# Autodesk Inventor assembly: Montagem do revórví
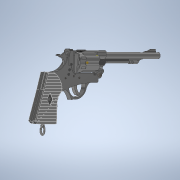
[picture p0: Inventor's stored thumbnail of the model, 180x180]
Saved by Autodesk Inventor 2021 (Build 250183000, 183)
## iProperties
Created: 2020-11-21
Part Number: Montagem do revórví
Document SubType Name: Assembly
Designer: Bruno
Author: Bruno
## Documents named in this file (20)
- C:\Users\Bruno\Documents\Quadirmestre Suplementar\Projeto Assistido por Computador\Novas peças revólver\Montagem do revórví.iam
- C:\Users\Bruno\Documents\Quadirmestre Suplementar\Projeto Assistido por Computador\Novas peças revólver\Part19.ipt
- C:\Users\Bruno\Documents\Quadirmestre Suplementar\Projeto Assistido por Computador\Novas peças revólver\Part22_1.ipt
- C:\Users\Bruno\Documents\Quadirmestre Suplementar\Projeto Assistido por Computador\Novas peças revólver\Part22_2.ipt
- C:\Users\Bruno\Documents\Quadirmestre Suplementar\Projeto Assistido por Computador\Novas peças revólver\Part35.ipt
- C:\Users\Bruno\Documents\Quadirmestre Suplementar\Projeto Assistido por Computador\Novas peças revólver\Montagem peças superiores.iam
- C:\Users\Bruno\Documents\Quadirmestre Suplementar\Projeto Assistido por Computador\Novas peças revólver\Montagem peças 11 a 14.iam
- C:\Users\Bruno\Documents\Quadirmestre Suplementar\Projeto Assistido por Computador\Novas peças revólver\Part6.ipt
- C:\Users\Bruno\Documents\Quadirmestre Suplementar\Projeto Assistido por Computador\Novas peças revólver\Montagem peças internas.iam
- C:\Users\Bruno\Documents\Quadirmestre Suplementar\Projeto Assistido por Computador\Novas peças revólver\Part41.ipt
- C:\Users\Bruno\Documents\Quadirmestre Suplementar\Projeto Assistido por Computador\Novas peças revólver\Part2.ipt
- C:\Users\Bruno\Documents\Quadirmestre Suplementar\Projeto Assistido por Computador\Novas peças revólver\Part37.ipt
- C:\Users\Bruno\Downloads\ECROU_M6_V1.ipt
- C:\Users\Bruno\Documents\Quadirmestre Suplementar\Projeto Assistido por Computador\Novas peças revólver\Parafuso_3mm.ipt
- C:\Users\Bruno\Documents\Quadirmestre Suplementar\Projeto Assistido por Computador\Novas peças revólver\Parafuso 2,031.ipt
- C:\Users\Bruno\Documents\Quadirmestre Suplementar\Projeto Assistido por Computador\Novas peças revólver\Parafuso15.ipt
- C:\Users\Bruno\Documents\Quadirmestre Suplementar\Projeto Assistido por Computador\Novas peças revólver\Parafuso1.5_2.ipt
- C:\Users\Bruno\Documents\Quadirmestre Suplementar\Projeto Assistido por Computador\Novas peças revólver\Parafuso 2_2 mm.ipt
- C:\Users\Bruno\Documents\Quadirmestre Suplementar\Projeto Assistido por Computador\Novas peças revólver\Parafuso1.5_3.ipt
- C:\Users\Bruno\Documents\Quadirmestre Suplementar\Projeto Assistido por Computador\Novas peças revólver\Parafuso 2_3 mm.ipt
## Components (21 placed, 19 different names)
1. Part19:1 — Rígida:5, Coincidente:16, Rotativa:1, Coincidente:17, Coincidente:20, Coincidente:21, Coincidente:27, Coincidente:28, Rígida:6, Plana:1, Coincidente:30, Coincidente:31, Coincidente:32, Coincidente:33, Coincidente:34, Coincidente:35, Coincidente:37, Coincidente:42, Coincidente:44, Alinhado:1, Coincidente:46, Coincidente:48, Coincidente:49, Coincidente:50, Coincidente:51, Coincidente:52, Coincidente:53, Coincidente:54, Coincidente:55
2. Part22_2:1 — Rígida:5
3. Montagem peças superiores:1 [sub-assembly] — Coincidente:16, Rotativa:1, Coincidente:18
4. Montagem peças 11 a 14:1 [sub-assembly] — Coincidente:17, Coincidente:18
5. Part35:1 — Coincidente:20, Coincidente:21, Coincidente:25, Coincidente:26, Coincidente:36
6. Part6:1 — Coincidente:25, Coincidente:26, Coincidente:27, Coincidente:56, Coincidente:57
7. Montagem peças internas:1 [sub-assembly] — Coincidente:28, Coincidente:29, Coincidente:45, Coincidente:47, Alinhado:2, Alinhado:3, Alinhado:4, Alinhado:5, Alinhado:6
8. Part22_1:1 — Coincidente:29, Rígida:6, Coincidente:38, Coincidente:39
9. Part41:1 — Plana:1, Coincidente:30, Coincidente:31, Coincidente:44
10. Part2:1 — Coincidente:32, Coincidente:35, Coincidente:40, Coincidente:41, Coincidente:43, Alinhado:1
11. Part37:1 — Coincidente:33, Coincidente:34
12. ECROU_M6_V1:1 — Coincidente:36, Coincidente:37
13. Parafuso_3mm:1 — Coincidente:38, Coincidente:39
14. Parafuso 2,031:1 — Coincidente:40, Coincidente:41
15. Parafuso 2,031:2 — Coincidente:42, Coincidente:43
16. Parafuso15:1 — Coincidente:45, Coincidente:46, Coincidente:47, Alinhado:2
17. Parafuso1.5_2:1 — Coincidente:48, Coincidente:49, Alinhado:3
18. Parafuso 2_2 mm:1 — Coincidente:50, Coincidente:51, Alinhado:4
19. Parafuso 2_2 mm:2 — Coincidente:52, Coincidente:53, Alinhado:5
20. Parafuso1.5_3:1 — Coincidente:54, Coincidente:55, Alinhado:6
21. Parafuso 2_3 mm:1 — Coincidente:56, Coincidente:57
## Relationships (48: Mate 38, Flush 6, WeldJoint 2, RevoluteJoint 1, PlanarJoint 1)
- Rígida:5 [WeldJoint]: Part19:1 ↔ Part22_2:1
- Coincidente:16 [Mate]: Part19:1 ↔ Montagem peças superiores:1
- Rotativa:1 [RevoluteJoint]: Part19:1 ↔ Montagem peças superiores:1
- Coincidente:17 [Mate]: Part19:1 ↔ Montagem peças 11 a 14:1
- Coincidente:18 [Mate]: Montagem peças superiores:1 ↔ Montagem peças 11 a 14:1
- Coincidente:20 [Mate]: Part19:1 ↔ Part35:1
- Coincidente:21 [Mate]: Part19:1 ↔ Part35:1
- Coincidente:25 [Mate]: Part35:1 ↔ Part6:1
- Coincidente:26 [Mate]: Part35:1 ↔ Part6:1
- Coincidente:27 [Mate]: Part19:1 ↔ Part6:1
- Coincidente:28 [Mate] (0.1 mm): Part19:1 ↔ Montagem peças internas:1
- Coincidente:29 [Mate]: Montagem peças internas:1 ↔ Part22_1:1
- Rígida:6 [WeldJoint]: Part19:1 ↔ Part22_1:1
- Plana:1: Part19:1 ↔ Part41:1
- Coincidente:30 [Mate]: Part19:1 ↔ Part41:1
- Coincidente:31 [Mate]: Part19:1 ↔ Part41:1
- Coincidente:32 [Mate]: Part19:1 ↔ Part2:1
- Coincidente:33 [Mate]: Part19:1 ↔ Part37:1
- Coincidente:34 [Mate]: Part19:1 ↔ Part37:1
- Coincidente:35 [Mate]: Part19:1 ↔ Part2:1
- Coincidente:36 [Mate]: Part35:1 ↔ ECROU_M6_V1:1
- Coincidente:37 [Mate]: Part19:1 ↔ ECROU_M6_V1:1
- Coincidente:38 [Mate]: Part22_1:1 ↔ Parafuso_3mm:1
- Coincidente:39 [Mate]: Part22_1:1 ↔ Parafuso_3mm:1
- Coincidente:40 [Mate]: Part2:1 ↔ Parafuso 2,031:1
- Coincidente:41 [Mate]: Part2:1 ↔ Parafuso 2,031:1
- Coincidente:42 [Mate]: Part19:1 ↔ Parafuso 2,031:2
- Coincidente:43 [Mate]: Part2:1 ↔ Parafuso 2,031:2
- Coincidente:44 [Mate]: Part19:1 ↔ Part41:1
- Alinhado:1 [Flush] (3.715 mm): Part19:1 ↔ Part2:1
- Coincidente:45 [Mate]: Montagem peças internas:1 ↔ Parafuso15:1
- Coincidente:46 [Mate]: Part19:1 ↔ Parafuso15:1
- Coincidente:47 [Mate]: Montagem peças internas:1 ↔ Parafuso15:1
- Alinhado:2 [Flush]: Montagem peças internas:1 ↔ Parafuso15:1
- Coincidente:48 [Mate]: Part19:1 ↔ Parafuso1.5_2:1
- Coincidente:49 [Mate]: Part19:1 ↔ Parafuso1.5_2:1
- Alinhado:3 [Flush]: Montagem peças internas:1 ↔ Parafuso1.5_2:1
- Coincidente:50 [Mate]: Part19:1 ↔ Parafuso 2_2 mm:1
- Coincidente:51 [Mate]: Part19:1 ↔ Parafuso 2_2 mm:1
- Alinhado:4 [Flush]: Montagem peças internas:1 ↔ Parafuso 2_2 mm:1
- Coincidente:52 [Mate]: Part19:1 ↔ Parafuso 2_2 mm:2
- Coincidente:53 [Mate]: Part19:1 ↔ Parafuso 2_2 mm:2
- Alinhado:5 [Flush]: Montagem peças internas:1 ↔ Parafuso 2_2 mm:2
- Coincidente:54 [Mate]: Part19:1 ↔ Parafuso1.5_3:1
- Coincidente:55 [Mate]: Part19:1 ↔ Parafuso1.5_3:1
- Alinhado:6 [Flush]: Montagem peças internas:1 ↔ Parafuso1.5_3:1
- Coincidente:56 [Mate]: Part6:1 ↔ Parafuso 2_3 mm:1
- Coincidente:57 [Mate]: Part6:1 ↔ Parafuso 2_3 mm:1
